# Autodesk Inventor assembly: VP-Dual-775pro
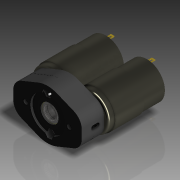
[picture p0: Inventor's stored thumbnail of the model, 180x180]
Saved by Autodesk Inventor 2022 (Build 260153000, 153)
## iProperties
Created: 2018-08-19
Part Number: VP-Dual-775pro
Document SubType Name: Assembly
Mass: 823.352 g
Surface Area: 940.04 cm^2
Volume: 140.134 cm^3
Density: 5.87546 g/cm^3
## Documents named in this file (15)
- E:\Middleton Robotics\Collaborative Robots\Collaborative Part Library\General Gearboxes\Planetaries\Versaplanetary\V2 Stages\Dual Input Stage\VP Dual 775pro Input.iam
- E:\Middleton Robotics\Collaborative Robots\Collaborative Part Library\General Gearboxes\Planetaries\Versaplanetary\V2 Stages\Dual Input Housing.ipt
- E:\Middleton Robotics\Collaborative Robots\Collaborative Part Library\General Gearboxes\Planetaries\Versaplanetary\V2 Stages\775pro Dual Input.ipt
- E:\Middleton Robotics\Collaborative Robots\Collaborative Part Library\General Gearboxes\Planetaries\Versaplanetary\V2 Stages\Dual Input Alignment Pin.ipt
- E:\Middleton Robotics\Collaborative Robots\Collaborative Part Library\General Gearboxes\Planetaries\Versaplanetary\Screws\8-32 Lock Nut.ipt
- E:\Middleton Robotics\Collaborative Robots\Collaborative Part Library\General Gearboxes\Planetaries\Versaplanetary\Screws\8-32 x 0.75in Screw.ipt
- E:\Middleton Robotics\Collaborative Robots\Collaborative Part Library\Motors\FRC\775pro.ipt
- E:\Middleton Robotics\Collaborative Robots\Collaborative Part Library\General Gearboxes\Planetaries\Versaplanetary\Screws\M4 x 10mm Screw.ipt
- E:\Middleton Robotics\Collaborative Robots\Collaborative Part Library\General Gearboxes\Planetaries\Versaplanetary\V2 Stages\Dual Input Output Gear.ipt
- E:\Middleton Robotics\Collaborative Robots\Collaborative Part Library\General Gearboxes\Planetaries\Versaplanetary\V2 Stages\Dual Input Coupler Gear.ipt
- E:\Middleton Robotics\Collaborative Robots\Collaborative Part Library\General Gearboxes\Planetaries\Versaplanetary\Input Coupler\5mm Coupler Sleeve.ipt
- E:\Middleton Robotics\Collaborative Robots\Collaborative Part Library\General Gearboxes\Planetaries\Versaplanetary\Input Coupler\Coupler Set Screw.ipt
- E:\Middleton Robotics\Collaborative Robots\Collaborative Part Library\Power Transfer\Bearings and Bushings\Bearings\6803ZZ.ipt
- E:\Middleton Robotics\Collaborative Robots\Collaborative Part Library\General Gearboxes\Planetaries\Versaplanetary\V2 Stages\Dual Input Stage.iam
- D:\FIRST\Design\CollabPartsLib\Power Transfer\Bearings.ipt
## Components (22 placed, 12 different names)
1. Dual Input Housing:1 — Insert:3, Mate:1, Mate:2, Insert:4, Angle:1, Insert:5, Angle:2, Mate:3, Mate:8, Mate:15, Insert:38, Mate:16, Flush:3, Flush:4, Insert:39, Mate:17
2. 6803ZZ:1 — Insert:36, Insert:38
3. 775pro Dual Input:1 — Mate:1, Mate:2, Insert:6, Insert:7, Insert:8, Insert:9, Insert:10, Insert:11, Insert:12, Insert:13, Insert:14, Mate:15
4. 6803ZZ:2 — Insert:37
5. Dual Input Alignment Pin:1 — Insert:3
6. 8-32 Lock Nut:1 — Insert:4, Angle:1
7. 8-32 Lock Nut:2 — Insert:5, Angle:2
8. 8-32 x 0.75in Screw:1 — Insert:6, Flush:1, Mate:8
9. 8-32 x 0.75in Screw:2 — Mate:3, Flush:1
10. 775pro:1 — Insert:7, Insert:8
11. 775pro:2 — Insert:9, Insert:10
12. M4 x 10mm Screw:1 — Insert:11
13. M4 x 10mm Screw:2 — Insert:12
14. M4 x 10mm Screw:3 — Insert:13
15. M4 x 10mm Screw:4 — Insert:14
16. Dual Input Output Gear:1 — Rotation:1, Rotation:2, Insert:36, Insert:37
17. Dual Input Coupler Gear:1 — Insert:19, Rotation:2, Angle:4, Mate:5, Tangent:2, Flush:2
18. Dual Input Coupler Gear:2 — Insert:18, Rotation:1, Angle:3, Mate:4, Tangent:1, Flush:2, Insert:39
19. 5mm Coupler Sleeve:1 — Insert:18, Angle:3
20. 5mm Coupler Sleeve:2 — Insert:19, Angle:4, Mate:17
21. Coupler Set Screw:1 — Mate:4, Tangent:1
22. Coupler Set Screw:2 — Mate:5, Tangent:2
## Relationships (39: Insert 18, Mate 9, Angle 4, Flush 4, RelateRotation 2, Tangent 2)
- Insert:3: Dual Input Housing:1 ↔ Dual Input Alignment Pin:1
- Mate:1: Dual Input Housing:1 ↔ 775pro Dual Input:1
- Mate:2: Dual Input Housing:1 ↔ 775pro Dual Input:1
- Insert:4: Dual Input Housing:1 ↔ 8-32 Lock Nut:1
- Angle:1 (0 deg): Dual Input Housing:1 ↔ 8-32 Lock Nut:1
- Insert:5: Dual Input Housing:1 ↔ 8-32 Lock Nut:2
- Angle:2 (0 deg): Dual Input Housing:1 ↔ 8-32 Lock Nut:2
- Insert:6: 775pro Dual Input:1 ↔ 8-32 x 0.75in Screw:1
- Mate:3: Dual Input Housing:1 ↔ 8-32 x 0.75in Screw:2
- Flush:1: 8-32 x 0.75in Screw:1 ↔ 8-32 x 0.75in Screw:2
- Insert:7: 775pro Dual Input:1 ↔ 775pro:1
- Insert:8: 775pro Dual Input:1 ↔ 775pro:1
- Insert:9: 775pro Dual Input:1 ↔ 775pro:2
- Insert:10: 775pro Dual Input:1 ↔ 775pro:2
- Insert:11: 775pro Dual Input:1 ↔ M4 x 10mm Screw:1
- Insert:12: 775pro Dual Input:1 ↔ M4 x 10mm Screw:2
- Insert:13: 775pro Dual Input:1 ↔ M4 x 10mm Screw:3
- Insert:14: 775pro Dual Input:1 ↔ M4 x 10mm Screw:4
- Insert:18: Dual Input Coupler Gear:2 ↔ 5mm Coupler Sleeve:1
- Insert:19: Dual Input Coupler Gear:1 ↔ 5mm Coupler Sleeve:2
- Rotation:1 [RelateRotation] (1 ul): Dual Input Output Gear:1 ↔ Dual Input Coupler Gear:2
- Rotation:2 [RelateRotation] (1 ul): Dual Input Output Gear:1 ↔ Dual Input Coupler Gear:1
- Angle:3 (0 deg): Dual Input Coupler Gear:2 ↔ 5mm Coupler Sleeve:1
- Angle:4 (0 deg): Dual Input Coupler Gear:1 ↔ 5mm Coupler Sleeve:2
- Mate:4: Dual Input Coupler Gear:2 ↔ Coupler Set Screw:1
- Tangent:1: Dual Input Coupler Gear:2 ↔ Coupler Set Screw:1
- Mate:5: Dual Input Coupler Gear:1 ↔ Coupler Set Screw:2
- Tangent:2: Dual Input Coupler Gear:1 ↔ Coupler Set Screw:2
- Mate:8: Dual Input Housing:1 ↔ 8-32 x 0.75in Screw:1
- Flush:2: Dual Input Coupler Gear:1 ↔ Dual Input Coupler Gear:2
- Mate:15: Dual Input Housing:1 ↔ 775pro Dual Input:1
- Insert:36: 6803ZZ:1 ↔ Dual Input Output Gear:1
- Insert:37: 6803ZZ:2 ↔ Dual Input Output Gear:1
- Insert:38: Dual Input Housing:1 ↔ 6803ZZ:1
- Mate:16: Dual Input Housing:1
- Flush:3: Dual Input Housing:1
- Flush:4: Dual Input Housing:1
- Insert:39: Dual Input Housing:1 ↔ Dual Input Coupler Gear:2
- Mate:17: Dual Input Housing:1 ↔ 5mm Coupler Sleeve:2
